# Autodesk Inventor assembly: extruderAssem
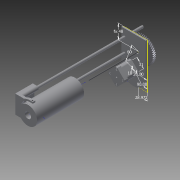
[picture p0: Inventor's stored thumbnail of the model, 180x180]
Saved by Autodesk Inventor 2015 SP2 (Build 190223200, 223)
## iProperties
Created: 2016-03-07
Part Number: extruderAssem
Document SubType Name: Assembly
Designer: marc
Author: marc
## Documents named in this file (11)
- C:\Users\marc\Documents\GitHub\Prusa_i3\Extruder\pusherDesign\extruderAssem.iam
- C:\Users\marc\Documents\GitHub\Prusa_i3\Extruder\pusherDesign\base.ipt
- C:\Users\marc\Documents\GitHub\Prusa_i3\Extruder\pusherDesign\rod.ipt
- C:\Users\marc\Documents\GitHub\Prusa_i3\Extruder\pusherDesign\CapHolder.ipt
- C:\Users\marc\Documents\GitHub\Prusa_i3\Extruder\pusherDesign\cylinder.ipt
- C:\Users\marc\Documents\GitHub\Prusa_i3\Extruder\pusherDesign\plate_bot.ipt
- C:\Users\marc\Documents\GitHub\Prusa_i3\Extruder\pusherDesign\threadedRod.ipt
- C:\Users\marc\Documents\GitHub\Prusa_i3\standard_parts\en-US\DIN 625 SKF(4)\DIN 625 SKF - SKF 608-2Z.ipt
- C:\Users\marc\Documents\GitHub\Prusa_i3\Imported Components\NEMA 17 Stepper Motor Assembly\NEMA 17 Stepper Motor Assembly.iam
- C:\Users\marc\Documents\GitHub\Prusa_i3\Extruder\pusherDesign\extruderAssem\Design Accelerator\Spur Gears3.iam
- C:\Users\marc\Documents\GitHub\Prusa_i3\standard_parts\en-US\ISO 7089\ISO 7089 - 6 - 140 HV(1).ipt
## Components (11 placed, 10 different names)
1. base:1 — Mate:1, Mate:2, Mate:3, Cylindrical:1, Cylindrical:2, Mate:4, Mate:5, Cylindrical:9, Mate:6, Angle:1
2. rod:1 — Cylindrical:2, Mate:5, Cylindrical:5
3. rod:2 — Cylindrical:1, Mate:4, Cylindrical:6
4. CapHolder:1 — Cylindrical:7, Cylindrical:8, Angle:1
5. cylinder:1 — Cylindrical:7, Cylindrical:8, Cylindrical:9, Mate:6
6. plate_bot:1 — Cylindrical:5, Cylindrical:6, Cylindrical:10, Mate:8, Mate:9, Cylindrical:11, Cylindrical:12
7. threadedRod:1 — Cylindrical:10, Mate:7, Mate:10, Cylindrical:13
8. DIN 625 SKF- with two Z shields SKF 608-2Z:1 — Mate:7, Mate:8, Mate:12
9. NEMA 17 Stepper Motor Assembly:1 [sub-assembly] — Mate:9, Cylindrical:11, Cylindrical:12, Mate:11
10. Spur Gears:1 [sub-assembly] — Mate:10, Mate:11, Mate:13
11. ISO 7089 6 - 140 HV:1 — Cylindrical:13, Mate:12, Mate:13
## Relationships (25: Mate 13, CylindricalJoint 11, Angle 1)
- Mate:1: base:1
- Mate:2: base:1
- Mate:3: base:1
- Cylindrical:1: base:1 ↔ rod:2
- Cylindrical:2: base:1 ↔ rod:1
- Mate:4: base:1 ↔ rod:2
- Mate:5: base:1 ↔ rod:1
- Cylindrical:5: rod:1 ↔ plate_bot:1
- Cylindrical:6: rod:2 ↔ plate_bot:1
- Cylindrical:7: CapHolder:1 ↔ cylinder:1
- Cylindrical:8: CapHolder:1 ↔ cylinder:1
- Cylindrical:9: base:1 ↔ cylinder:1
- Mate:6: base:1 ↔ cylinder:1
- Angle:1 (0 deg): base:1 ↔ CapHolder:1
- Cylindrical:10: plate_bot:1 ↔ threadedRod:1
- Mate:7: threadedRod:1 ↔ DIN 625 SKF- with two Z shields SKF 608-2Z:1
- Mate:8: plate_bot:1 ↔ DIN 625 SKF- with two Z shields SKF 608-2Z:1
- Mate:9: plate_bot:1 ↔ NEMA 17 Stepper Motor Assembly:1
- Cylindrical:11: plate_bot:1 ↔ NEMA 17 Stepper Motor Assembly:1
- Cylindrical:12: plate_bot:1 ↔ NEMA 17 Stepper Motor Assembly:1
- Mate:10: threadedRod:1 ↔ Spur Gears:1
- Mate:11: NEMA 17 Stepper Motor Assembly:1 ↔ Spur Gears:1
- Cylindrical:13: threadedRod:1 ↔ ISO 7089 6 - 140 HV:1
- Mate:12: DIN 625 SKF- with two Z shields SKF 608-2Z:1 ↔ ISO 7089 6 - 140 HV:1
- Mate:13: Spur Gears:1 ↔ ISO 7089 6 - 140 HV:1
